# Autodesk Inventor assembly: EyasSay_Ensamblaje
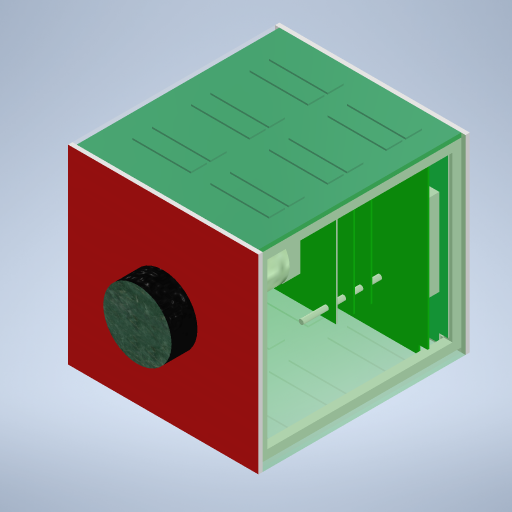
[picture p0: Inventor's stored thumbnail of the model, 512x512]
Saved by Autodesk Inventor 2024 (Build 280153000, 153)
## iProperties
Created: 2023-06-26
Part Number: EyasSay_Ensamblaje
Document SubType Name: Assembly
Designer: Personal
Mass: 3302.12 g
Surface Area: 8181.14 cm^2
Volume: 1723.1 cm^3
Density: 1.91638 g/cm^3
Author: Personal
## Documents named in this file (15)
- D:\Personal\Documents\GitHub\TDG_ReactionWheelsUnloading\Inventor\EyasSat_medicionesReales\EyasSay_Ensamblaje_rotacion.iam
- D:\Personal\Documents\GitHub\TDG_ReactionWheelsUnloading\Inventor\EyasSat_medicionesReales\Acrilico_Bottom.ipt
- D:\Personal\Documents\GitHub\TDG_ReactionWheelsUnloading\Inventor\EyasSat_medicionesReales\AcrilicoX.ipt
- D:\Personal\Documents\GitHub\TDG_ReactionWheelsUnloading\Inventor\EyasSat_medicionesReales\AcrilicoX_MIR.ipt
- D:\Personal\Documents\GitHub\TDG_ReactionWheelsUnloading\Inventor\EyasSat_medicionesReales\AcrilicoY.ipt
- D:\Personal\Documents\GitHub\TDG_ReactionWheelsUnloading\Inventor\EyasSat_medicionesReales\AcrilicoY_MIR.ipt
- D:\Personal\Documents\GitHub\TDG_ReactionWheelsUnloading\Inventor\EyasSat_medicionesReales\BarraVertical.ipt
- D:\Personal\Documents\GitHub\TDG_ReactionWheelsUnloading\Inventor\EyasSat_medicionesReales\BarraVertical_MIR.ipt
- D:\Personal\Documents\GitHub\TDG_ReactionWheelsUnloading\Inventor\EyasSat_medicionesReales\BarraVertical_MIR1.ipt
- D:\Personal\Documents\GitHub\TDG_ReactionWheelsUnloading\Inventor\EyasSat_medicionesReales\BarraVertical_MIR_MIR.ipt
- D:\Personal\Documents\GitHub\TDG_ReactionWheelsUnloading\Inventor\EyasSat_medicionesReales\PCB_COM_BAT.ipt
- D:\Personal\Documents\GitHub\TDG_ReactionWheelsUnloading\Inventor\EyasSat_medicionesReales\Baterias\BATTERY HOLDER x2 18650\BATTERY HOLDER x2 18650.ipt
- D:\Personal\Documents\GitHub\TDG_ReactionWheelsUnloading\Inventor\EyasSat_medicionesReales\PCB_RW.ipt
- D:\Personal\Documents\GitHub\TDG_ReactionWheelsUnloading\Inventor\EyasSat_medicionesReales\Acrilico_Top.ipt
- D:\Personal\Documents\GitHub\TDG_ReactionWheelsUnloading\Inventor\EyasSat_medicionesReales\BarraHorizontal.ipt
## Components (17 placed, 14 different names)
1. Acrilico_Bottom:1 — Coincidencia:1, Coincidencia:2, Coincidencia:3, Coincidencia:4, Nivelación:1, Nivelación:2, Coincidencia:5, Nivelación:3, Nivelación:4, Nivelación:5, Nivelación:6, Nivelación:7, Nivelación:9, Nivelación:10, Coincidencia:9, Nivelación:24, Nivelación:25, Coincidencia:32, Coincidencia:33, Coincidencia:34, Coincidencia:35, Coincidencia:36, Coincidencia:37
2. AcrilicoX:1 — Coincidencia:4, Nivelación:1, Nivelación:2, Coincidencia:10, Nivelación:17, Coincidencia:18
3. AcrilicoX_MIR:1 — Coincidencia:5, Nivelación:3, Nivelación:4, Coincidencia:6, Coincidencia:15, Coincidencia:17
4. AcrilicoY:1 — Nivelación:5, Nivelación:6, Coincidencia:6, Nivelación:7, Nivelación:18
5. AcrilicoY_MIR:1 — Coincidencia:16, Coincidencia:17, Coincidencia:18, Nivelación:19, Coincidencia:27
6. BarraVertical:1 — Nivelación:9, Nivelación:10, Coincidencia:9, Coincidencia:10, Coincidencia:25, Coincidencia:27, Coincidencia:30, Nivelación:23
7. BarraVertical_MIR:1 — Coincidencia:22, Coincidencia:28, Nivelación:22, Nivelación:24, Nivelación:25, Coincidencia:32
8. BarraVertical_MIR1:1 — Coincidencia:21, Coincidencia:29
9. BarraVertical_MIR_MIR:1 — Coincidencia:19, Coincidencia:24, Nivelación:20, Nivelación:21
10. PCB_COM_BAT:1 — Coincidencia:33, Coincidencia:34, Coincidencia:35, Coincidencia:38, Coincidencia:39, Coincidencia:41
11. BATTERY HOLDER x2 18650:1 — Coincidencia:39, Coincidencia:40, Coincidencia:41
12. PCB_RW:1 — Nivelación:15, Nivelación:16, Coincidencia:36, Coincidencia:37, Coincidencia:38
13. Acrilico_Top:1 — Coincidencia:15, Nivelación:17, Nivelación:18, Coincidencia:16, Nivelación:19, Coincidencia:20, Coincidencia:23, Coincidencia:26, Coincidencia:31, Nivelación:26
14. BarraHorizontal:1 — Coincidencia:19, Coincidencia:20, Coincidencia:21, Nivelación:20
15. BarraHorizontal:2 — Coincidencia:25, Coincidencia:26, Coincidencia:28, Nivelación:22
16. BarraHorizontal:3 — Coincidencia:29, Coincidencia:30, Nivelación:23, Coincidencia:31
17. BarraHorizontal:4 — Coincidencia:22, Coincidencia:23, Coincidencia:24, Nivelación:21, Nivelación:26
## Relationships (56: Mate 35, Flush 21)
- Coincidencia:1 [Mate] (-106 mm): Acrilico_Bottom:1
- Coincidencia:2 [Mate] (-97.5 mm): Acrilico_Bottom:1
- Coincidencia:3 [Mate] (-97.5 mm): Acrilico_Bottom:1
- Coincidencia:4 [Mate]: Acrilico_Bottom:1 ↔ AcrilicoX:1
- Nivelación:1 [Flush]: Acrilico_Bottom:1 ↔ AcrilicoX:1
- Nivelación:2 [Flush]: Acrilico_Bottom:1 ↔ AcrilicoX:1
- Coincidencia:5 [Mate]: Acrilico_Bottom:1 ↔ AcrilicoX_MIR:1
- Nivelación:3 [Flush]: Acrilico_Bottom:1 ↔ AcrilicoX_MIR:1
- Nivelación:4 [Flush]: Acrilico_Bottom:1 ↔ AcrilicoX_MIR:1
- Nivelación:5 [Flush]: Acrilico_Bottom:1 ↔ AcrilicoY:1
- Nivelación:6 [Flush]: Acrilico_Bottom:1 ↔ AcrilicoY:1
- Coincidencia:6 [Mate]: AcrilicoX_MIR:1 ↔ AcrilicoY:1
- Nivelación:7 [Flush]: Acrilico_Bottom:1 ↔ AcrilicoY:1
- Nivelación:9 [Flush]: Acrilico_Bottom:1 ↔ BarraVertical:1
- Nivelación:10 [Flush]: Acrilico_Bottom:1 ↔ BarraVertical:1
- Coincidencia:9 [Mate]: Acrilico_Bottom:1 ↔ BarraVertical:1
- Coincidencia:10 [Mate]: AcrilicoX:1 ↔ BarraVertical:1
- Nivelación:15 [Flush]: PCB_RW:1
- Nivelación:16 [Flush]: PCB_RW:1
- Coincidencia:15 [Mate]: AcrilicoX_MIR:1 ↔ Acrilico_Top:1
- Nivelación:17 [Flush]: AcrilicoX:1 ↔ Acrilico_Top:1
- Nivelación:18 [Flush]: AcrilicoY:1 ↔ Acrilico_Top:1
- Coincidencia:16 [Mate]: AcrilicoY_MIR:1 ↔ Acrilico_Top:1
- Coincidencia:17 [Mate]: AcrilicoX_MIR:1 ↔ AcrilicoY_MIR:1
- Coincidencia:18 [Mate]: AcrilicoX:1 ↔ AcrilicoY_MIR:1
- Nivelación:19 [Flush]: AcrilicoY_MIR:1 ↔ Acrilico_Top:1
- Coincidencia:19 [Mate]: BarraVertical_MIR_MIR:1 ↔ BarraHorizontal:1
- Coincidencia:20 [Mate]: Acrilico_Top:1 ↔ BarraHorizontal:1
- Coincidencia:21 [Mate]: BarraVertical_MIR1:1 ↔ BarraHorizontal:1
- Coincidencia:22 [Mate]: BarraVertical_MIR:1 ↔ BarraHorizontal:4
- Coincidencia:23 [Mate]: Acrilico_Top:1 ↔ BarraHorizontal:4
- Coincidencia:24 [Mate]: BarraVertical_MIR_MIR:1 ↔ BarraHorizontal:4
- Nivelación:20 [Flush]: BarraVertical_MIR_MIR:1 ↔ BarraHorizontal:1
- Nivelación:21 [Flush]: BarraVertical_MIR_MIR:1 ↔ BarraHorizontal:4
- Coincidencia:25 [Mate]: BarraVertical:1 ↔ BarraHorizontal:2
- Coincidencia:26 [Mate]: Acrilico_Top:1 ↔ BarraHorizontal:2
- Coincidencia:27 [Mate]: AcrilicoY_MIR:1 ↔ BarraVertical:1
- Coincidencia:28 [Mate]: BarraVertical_MIR:1 ↔ BarraHorizontal:2
- Nivelación:22 [Flush]: BarraVertical_MIR:1 ↔ BarraHorizontal:2
- Coincidencia:29 [Mate]: BarraVertical_MIR1:1 ↔ BarraHorizontal:3
- Coincidencia:30 [Mate]: BarraVertical:1 ↔ BarraHorizontal:3
- Nivelación:23 [Flush]: BarraVertical:1 ↔ BarraHorizontal:3
- Coincidencia:31 [Mate]: Acrilico_Top:1 ↔ BarraHorizontal:3
- Nivelación:24 [Flush]: Acrilico_Bottom:1 ↔ BarraVertical_MIR:1
- Nivelación:25 [Flush]: Acrilico_Bottom:1 ↔ BarraVertical_MIR:1
- Coincidencia:32 [Mate]: Acrilico_Bottom:1 ↔ BarraVertical_MIR:1
- Coincidencia:33 [Mate]: Acrilico_Bottom:1 ↔ PCB_COM_BAT:1
- Coincidencia:34 [Mate]: Acrilico_Bottom:1 ↔ PCB_COM_BAT:1
- Coincidencia:35 [Mate]: Acrilico_Bottom:1 ↔ PCB_COM_BAT:1
- Coincidencia:36 [Mate]: Acrilico_Bottom:1 ↔ PCB_RW:1
- Coincidencia:37 [Mate]: Acrilico_Bottom:1 ↔ PCB_RW:1
- Coincidencia:38 [Mate] (16 mm): PCB_COM_BAT:1 ↔ PCB_RW:1
- Coincidencia:39 [Mate]: PCB_COM_BAT:1 ↔ BATTERY HOLDER x2 18650:1
- Coincidencia:40 [Mate]: BATTERY HOLDER x2 18650:1
- Coincidencia:41 [Mate] (-79 mm): PCB_COM_BAT:1 ↔ BATTERY HOLDER x2 18650:1
- Nivelación:26 [Flush]: Acrilico_Top:1 ↔ BarraHorizontal:4
## Named parameters: Finish10_Area = 38.4845, Finish11_Area = 722.015, Finish11_Thickness = 0.05 mm, Finish1_Area = 617.392, Finish2_Area = 69.0691, Finish3_Area = 71.245, Finish4_Area = 12.5343, Finish5_Area = 61.0286, Finish6_Area = 51.4279, Finish7_Area = 341.765, Finish8_Area = 341.765, Finish9_Area = 438.527
note: some values were not read from the file. Shown as the stored number, unit unknown: "Finish10_Area", "Finish11_Area", "Finish1_Area", "Finish2_Area", "Finish3_Area", "Finish4_Area", "Finish5_Area", "Finish6_Area", "Finish7_Area", "Finish8_Area", "Finish9_Area".
